# Autodesk Inventor assembly: FullCartV1
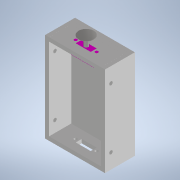
[picture p0: Inventor's stored thumbnail of the model, 180x180]
Saved by Autodesk Inventor 2020 (Build 240168000, 168)
## iProperties
Created: 2020-06-07
Part Number: FullCartV1
Document SubType Name: Assembly
Designer: Kitte_x
Author: Kitte_x
## Documents named in this file (7)
- C:\Users\Kitte_x\Documents\Inventor\Collison_Cart\FullCartV1.iam
- C:\Users\Kitte_x\Documents\Inventor\Collison_Cart\SideV1.ipt
- C:\Users\Kitte_x\Documents\Inventor\Collison_Cart\TopHolderV1.ipt
- C:\Users\Kitte_x\Documents\Inventor\Collison_Cart\TopPlateV1.ipt
- C:\Users\Kitte_x\Documents\Inventor\Collison_Cart\FrameV1.ipt
- C:\Users\Kitte_x\Documents\Inventor\Collison_Cart\SpringHolderV1.ipt
- C:\Users\Kitte_x\Documents\Inventor\Collison_Cart\SpringCapV1.ipt
## Components (8 placed, 6 different names)
1. SideV1:1 — Mate:1, Mate:4, Mate:5, Mate:6, Mate:7, Mate:11
2. TopHolderV1:1 — Mate:1, Mate:2, Mate:3, Mate:4, Mate:8
3. TopPlateV1:1 — Mate:5, Mate:6, Mate:7, Mate:8, Mate:9, Mate:10, Flush:1, Flush:2, Mate:13
4. SideV1:2 — Mate:2, Mate:3, Mate:9, Mate:12
5. FrameV1:1 — Mate:10, Mate:11, Flush:1, Flush:3, Mate:14, Mate:15
6. FrameV1:2 — Flush:2, Mate:12, Mate:13
7. SpringHolderV1:1 — Flush:3, Mate:14, Mate:15, Mate:16
8. SpringCapV1:1 — Mate:16
## Relationships (19: Mate 16, Flush 3)
- Mate:1: SideV1:1 ↔ TopHolderV1:1
- Mate:2: TopHolderV1:1 ↔ SideV1:2
- Mate:3: TopHolderV1:1 ↔ SideV1:2
- Mate:4: SideV1:1 ↔ TopHolderV1:1
- Mate:5: SideV1:1 ↔ TopPlateV1:1
- Mate:6: SideV1:1 ↔ TopPlateV1:1
- Mate:7: SideV1:1 ↔ TopPlateV1:1
- Mate:8: TopHolderV1:1 ↔ TopPlateV1:1
- Mate:9: TopPlateV1:1 ↔ SideV1:2
- Mate:10: TopPlateV1:1 ↔ FrameV1:1
- Mate:11: SideV1:1 ↔ FrameV1:1
- Flush:1: TopPlateV1:1 ↔ FrameV1:1
- Flush:2: TopPlateV1:1 ↔ FrameV1:2
- Mate:12: SideV1:2 ↔ FrameV1:2
- Mate:13: TopPlateV1:1 ↔ FrameV1:2
- Flush:3: FrameV1:1 ↔ SpringHolderV1:1
- Mate:14: FrameV1:1 ↔ SpringHolderV1:1
- Mate:15: FrameV1:1 ↔ SpringHolderV1:1
- Mate:16: SpringHolderV1:1 ↔ SpringCapV1:1
